# Autodesk Inventor assembly: gasienica_zlozenie
(part 2 of 2)
- [Mate]: ramie_2_wahacza:10 ↔ tuleja_TUF106040:39
- [Angle] (0 deg): ramie_2_wahacza:10 ↔ tuleja_TUF106040:39
- [Mate]: Korpus:5 ↔ Tlok:5
- [Angle] (0 deg): Korpus:5 ↔ Tlok:5
- [Mate]: Korpus:5 ↔ Nakretka:5
- [Mate] (5 mm): Korpus:5 ↔ Nakretka:5
- Walcowe:5 [CylindricalJoint]: Korpus:5 ↔ Tlok:5
- [Mate]: Korpus:5 ↔ M5_70_shaft:5
- [Flush] (-30 mm): Korpus:5 ↔ M5_70_shaft:5
- [Mate]: M5_nut_5mm:28 ↔ M5_70_shaft:5
- [Mate]: M5_70_shaft:5 ↔ M5_nut_5mm:29
- [Mate] (60 mm): M5_nut_5mm:28 ↔ M5_nut_5mm:29
- [Mate] (30 mm): Korpus:5 ↔ M5_nut_5mm:28
- [Mate]: tuleja_TUF106040:38 ↔ ramie_1_wahacza:10
- [Mate]: tuleja_TUF106040:37 ↔ ramie_1_wahacza:10
- [Mate]: tuleja_TUF106040:38 ↔ ramie_1_wahacza:10
- [Mate]: tuleja_TUF106040:33 ↔ tuleja_TUF106040:39
- [Mate]: wspornik_amortyzatora:9 ↔ wspornik_amortyzatora:10
- [Mate]: wspornik_amortyzatora:9 ↔ wspornik_amortyzatora:10
- [Mate] (5 mm): wspornik_amortyzatora:9 ↔ wspornik_amortyzatora:10
- [Mate]: M3_16_shaft:5 ↔ wspornik_amortyzatora:10
- [Flush] (-2.5 mm): M3_16_shaft:5 ↔ wspornik_amortyzatora:9
- [Mate]: M3_16_shaft:5 ↔ M3_nut_2,5mm:9
- [Mate]: M3_nut_2,5mm:9 ↔ wspornik_amortyzatora:9
- [Mate]: M3_16_shaft:5 ↔ M3_nut_2,5mm:10
- [Mate]: M3_nut_2,5mm:10 ↔ wspornik_amortyzatora:10
- [Mate]: Tlok:5 ↔ M3_16_shaft:5
- [Mate]: Tlok:5 ↔ wspornik_amortyzatora:10
- [Mate]: ramie_1_wahacza:9 ↔ wspornik_amortyzatora:9
- [Mate]: ramie_1_wahacza:9 ↔ wspornik_amortyzatora:9
- [Mate] (4.5 mm): ramie_1_wahacza:9 ↔ wspornik_amortyzatora:9
- [Mate]: tuleja_TUF106040:36 ↔ M6_40_shaft:9
- [Flush] (7 mm): ramie_1_wahacza:9 ↔ M6_40_shaft:9
- [Mate]: tuleja_TUF106040:39 ↔ M6_40_shaft:10
- [Flush] (7 mm): ramie_2_wahacza:10 ↔ M6_40_shaft:10
- [Mate]: M6_nut_5mm:41 ↔ M6_40_shaft:9
- [Mate]: ramie_1_wahacza:9 ↔ M6_nut_5mm:41
- [Mate]: M6_40_shaft:9 ↔ M6_nut_5mm:42
- [Mate]: ramie_1_wahacza:10 ↔ M6_nut_5mm:42
- [Mate]: M6_40_shaft:10 ↔ M6_nut_5mm:43
- [Mate]: ramie_2_wahacza:9 ↔ M6_nut_5mm:43
- [Mate]: M6_40_shaft:10 ↔ M6_nut_5mm:44
- [Mate]: ramie_2_wahacza:10 ↔ M6_nut_5mm:44
- [Mate]: M6_40_shaft:9 ↔ tuleja_M6_M10_7:10
- [Mate]: M6_40_shaft:10 ↔ tuleja_M6_M10_7:11
- [Mate]: M6_1,25_pad:33 ↔ M6_1,25_pad:34
- [Mate]: M6_1,25_pad:33 ↔ M6_1,25_pad:34
- [Mate]: M6_40_shaft:9 ↔ M6_1,25_pad:33
- [Mate]: M6_1,25_pad:35 ↔ M6_1,25_pad:36
- [Mate]: M6_1,25_pad:35 ↔ M6_1,25_pad:36
- [Mate]: M6_40_shaft:9 ↔ M6_1,25_pad:35
- [Mate]: tuleja_TUF106040:36 ↔ M6_1,25_pad:35
- [Mate]: M6_1,25_pad:37 ↔ M6_1,25_pad:38
- [Mate]: M6_1,25_pad:37 ↔ M6_1,25_pad:38
- [Mate]: M6_40_shaft:10 ↔ M6_1,25_pad:37
- [Mate]: M6_1,25_pad:39 ↔ M6_1,25_pad:40
- [Mate]: M6_1,25_pad:39 ↔ M6_1,25_pad:40
- [Mate]: M6_40_shaft:10 ↔ M6_1,25_pad:39
- [Mate]: tuleja_TUF106040:39 ↔ M6_1,25_pad:39
- [Mate]: M5_70_shaft:5 ↔ M6_70_shaft:9
- [Flush]: M5_70_shaft:5 ↔ M6_70_shaft:10
- [Mate]: M6_70_shaft:10 ↔ M6_nut_5mm:45
- [Mate]: M6_70_shaft:10 ↔ M6_nut_5mm:46
- [Mate] (60 mm): M6_nut_5mm:45 ↔ M6_nut_5mm:46
- [Flush]: M5_nut_5mm:28 ↔ M6_nut_5mm:46
- [Mate] (60 mm): M6_nut_5mm:47 ↔ M6_nut_5mm:48
- [Mate]: M6_nut_5mm:47 ↔ M6_nut_5mm:48
- [Mate]: M6_70_shaft:9 ↔ M6_nut_5mm:47
- [Flush]: M5_nut_5mm:28 ↔ M6_nut_5mm:48
- [Mate]: ramie_1_wahacza:9 ↔ M5_shaft:9
- [Flush] (7 mm): ramie_1_wahacza:9 ↔ M5_shaft:9
- [Mate]: ramie_1_wahacza:9 ↔ M5_shaft:10
- [Flush] (7 mm): ramie_1_wahacza:9 ↔ M5_shaft:10
- [Mate]: M5_shaft:10 ↔ M5_nut_5mm:30
- [Mate]: ramie_1_wahacza:9 ↔ M5_nut_5mm:30
- [Mate]: M5_shaft:9 ↔ M5_nut_5mm:31
- [Mate]: ramie_1_wahacza:9 ↔ M5_nut_5mm:31
- [Mate]: M5_shaft:9 ↔ M5_nut_5mm:32
- [Mate]: ramie_1_wahacza:10 ↔ M5_nut_5mm:32
- [Mate]: M5_shaft:10 ↔ M5_nut_5mm:33
- [Mate]: ramie_1_wahacza:10 ↔ M5_nut_5mm:33
- [Mate]: M5_70_shaft:5 ↔ tuleja_M5_M9_20:5
- [Mate]: Korpus:5 ↔ tuleja_M5_M9_20:5
- [Mate]: M5_70_shaft:5 ↔ tuleja_M5_M9_25:5
- [Mate]: Korpus:5 ↔ tuleja_M5_M9_25:5
- [Mate]: M5_shaft:9 ↔ tuleja_M5_M9_4,5:17
- [Mate]: ramie_1_wahacza:10 ↔ tuleja_M5_M9_4,5:17
- [Mate]: M5_shaft:9 ↔ tuleja_M5_M9_4,5:18
- [Mate]: ramie_1_wahacza:9 ↔ tuleja_M5_M9_4,5:18
- [Mate]: M5_shaft:10 ↔ tuleja_M5_M9_4,5:19
- [Mate]: ramie_1_wahacza:10 ↔ tuleja_M5_M9_4,5:19
- [Mate]: M5_shaft:10 ↔ tuleja_M5_M9_4,5:20
- [Mate]: ramie_1_wahacza:9 ↔ tuleja_M5_M9_4,5:20
- [Mate]: M6_40_shaft:10 ↔ glowny_wahacz_zewn:3
- [Mate]: tuleja_M6_M10_7:11 ↔ glowny_wahacz_zewn:3
- [Mate]: M6_40_shaft:9 ↔ glowny_wahacz_zewn:3
- [Mate]: M6_40_shaft:10 ↔ glowny_wahacz_zewn:4
- [Mate]: M6_40_shaft:9 ↔ glowny_wahacz_zewn:4
- [Mate]: tuleja_TUF106040:38 ↔ M6_40_shaft:9
- [Mate]: M6_1,25_pad:36 ↔ glowny_wahacz_zewn:4
- [Mate]: M6_1,25_pad:40 ↔ glowny_wahacz_zewn:4
- [Mate]: tuleja_M6_M10_7:10 ↔ glowny_wahacz_zewn:3
- [Mate]: M6_1,25_pad:33 ↔ glowny_wahacz_zewn:3
- [Mate]: tuleja_TUF106040:38 ↔ M6_1,25_pad:34
- [Mate]: M6_1,25_pad:37 ↔ glowny_wahacz_zewn:3
- [Mate]: tuleja_TUF106040:33 ↔ M6_1,25_pad:38
- [Mate]: tuleja_TUF106040:37 ↔ ramie_1_wahacza:10
- [Mate]: tuleja_TUF106040:35 ↔ M6_70_shaft:10
- [Mate]: ramie_1_wahacza:9 ↔ tuleja_TUF106040:35
- [Mate]: ramie_1_wahacza:9 ↔ tuleja_TUF106040:35
- [Mate]: tuleja_TUF106040:34 ↔ M6_70_shaft:9
- [Mate]: ramie_2_wahacza:9 ↔ tuleja_TUF106040:34
- [Mate]: ramie_2_wahacza:9 ↔ tuleja_TUF106040:34
- [Mate]: tuleja_TUF106040:40 ↔ M6_70_shaft:9
- [Mate]: ramie_2_wahacza:10 ↔ tuleja_TUF106040:40
- [Mate]: ramie_2_wahacza:10 ↔ tuleja_TUF106040:40
- [Mate]: M6_70_shaft:9 ↔ tuleja_M6_M10_8,5:9
- [Mate]: tuleja_TUF106040:40 ↔ tuleja_M6_M10_8,5:9
- [Mate]: M6_70_shaft:9 ↔ tuleja_M6_M10_13,5:9
- [Mate]: M6_70_shaft:10 ↔ tuleja_M6_M10_13,5:10
- [Mate]: tuleja_TUF106040:37 ↔ tuleja_M6_M10_13,5:10
- [Mate]: tuleja_TUF106040:34 ↔ tuleja_M6_M10_13,5:9
- [Mate]: M6_70_shaft:10 ↔ tuleja_M6_M10_8,5:10
- [Mate]: tuleja_TUF106040:35 ↔ tuleja_M6_M10_8,5:10
- [Mate]: independent_wheel_pair:2 ↔ tuleja_M6_M10_7:12
- [Mate]: glowny_wahacz_zewn:4 ↔ independent_wheel_pair:2
- [Mate]: glowny_wahacz_zewn:4 ↔ independent_wheel_pair:2
- [Mate]: glowny_wahacz_zewn:4 ↔ tuleja_M6_M10_7:12
- Zestawiające:1006 [Mate]: plyta_glowna_V3:2 ↔ M5_nut_5mm:28
- Zestawiające:1007 [Mate]: glowny_wahacz_zewn:3 ↔ independent_wheel_pair:2
- Zestawiające:1008 [Mate]: glowny_wahacz_zewn:3 ↔ tuleja_M6_M10_7:12
- Zestawiające:1009 [Mate]: plyta_glowna_V3:2 ↔ M6_70_shaft:10
- Zestawiające:1010 [Mate]: tuleja_TUF106040:37 ↔ M6_70_shaft:10
- Zestawiające:1011 [Mate]: plyta_glowna_V3:2 ↔ tuleja_M6_M10_13,5:9
- Zestawiające:1012 [Mate]: plyta_glowna_V3:2 ↔ tuleja_M5_M9_25:5
## Named parameters: d47_d24 = 0 mm, d48_d25 = 0 mm, d17_d47_d24 = 0 mm, d18_d48_d25 = 0 mm, d19_d15 = 0 mm, d20_d16 = 5 mm, d25_d17_d47_d24 = 0 mm, d26_d18_d48_d25 = 0 mm, d27_d19_d15 = 0 mm, d28_d20_d16 = 5 mm, d102_d31 = 0 mm, d103_d32 = 7 mm, d104_d33 = 0 mm, d105_d34 = 0 mm, d705_d35 = 0 mm, d706_d36 = 31 mm, d707_d37 = 0 mm, d109_d23 = 0 mm, d110_d24 = 0 mm, d111_d25 = 0 mm, d112_d26 = 0 mm, d113_d27 = 7 mm, d114_d28 = 0 mm, d115_d30 = 0 mm, d715_d116 = 0 mm, d716_d117 = 0 mm, d717_d118 = 0 mm, d718_d119 = 0 mm, susp_angle = 108 deg, d917_d233 = 0 mm, d918_d234 = 0 mm, d919_d235 = 0 mm, d920_d236 = 0 mm, d921_d237 = 0 mm, d922_d205 = 0 mm, d923_d206 = 0 mm, d924_d207 = 0 mm, d925_d208 = 0 mm, d926_d209 = 0 mm, d927_d210 = 0 mm, d928_d211 = 0 mm, d929_d212 = 0 mm, d930_d213 = 0 mm, d931_d214 = 0 mm, d932_d215 = 0 mm, d933_d216 = 0 mm, d934_d217 = 0 mm, d935_d218 = 0 mm, d936_d219 = 0 mm, d937_d220 = 0 mm, d938_d221 = 0 mm, d939_d222 = 0 mm, d940_d223 = 0 mm, d941_d224 = 0 mm, d942_d225 = 0 mm, d943_d226 = 0 mm, d944_d227 = 0 mm, d945_d228 = 0 mm, d946_d229 = 0 mm, d947_d230 = 0 mm, d948_d231 = 0 mm, d949_d232 = 0 mm, d950_d168 = 0 mm, d951_d169 = 0 mm, d952_d172 = 0 mm, d953_d173 = 0 mm, d954_d174 = 0 mm, d955_d175 = 0 mm, d956_d176 = 60 mm, d957_d177 = 0 mm, d958_d178_d176 = 60 mm, d959_d179 = 0 mm, d960_d180 = 0 mm, d961_d181 = 0 mm, d962_d190 = 0 mm, d963_d191 = 7 mm, d964_d192 = 0 mm, d965_d193 = 7 mm, d966_d194 = 0 mm, d967_d195 = 0 mm, d968_d196 = 0 mm, d969_d197 = 0 mm, d970_d198 = 0 mm, d971_d199 = 0 mm, d972_d200 = 0 mm, d973_d201 = 0 mm, d974_d202 = 0 mm, d975_d203 = 0 mm, d976_d204 = 0 mm, d977_d136 = 0 mm, d978_d137 = 4.5 mm, d979_d138 = 0 mm, d980_d139 = 7 mm, d981_d140 = 0 mm, d982_d141 = 7 mm, d983_d142 = 0 mm, d984_d143 = 0 mm, d985_d144 = 0 mm, d986_d145 = 0 mm, d987_d146 = 0 mm, d988_d147 = 0 mm, d989_d148 = 0 mm, d990_d149 = 0 mm, d991_d150 = 0 mm, d992_d151 = 0 mm, d993_d152 = 0 mm, d994_d153 = 0 mm, d995_d154 = 0 mm, d996_d155 = 0 mm, d997_d156 = 0 mm, d998_d157 = 0 mm, d999_d158_d154 = 0 mm, d1000_d159_d155 = 0 mm, d1001_d160 = 0 mm, d1002_d161 = 0 mm, d1003_d162_d154 = 0 mm, d1004_d163_d155 = 0 mm, d1005_d164 = 0 mm, d1006_d165 = 0 mm, d1007_d166_d154 = 0 mm, d1008_d167_d155 = 0 mm, d1009_d106 = 0 mm, d1010_d107 = 0 mm, d1011_d108 = 0 mm, d1012_d109 = -30 mm, d1013_d110 = 0 mm, d1014_d111 = 0 mm, d1015_d112 = 60 mm, d1016_d113 = 30 mm, d1017_d114 = 0 mm, d1018_d116 = 0 mm, d1019_d118 = 0 mm, d1020_d119 = 0 mm, d1021_d120 = 0 mm, d1022_d121 = 0 mm, d1023_d122 = 5 mm, d1024_d123 = 0 mm, d1025_d124 = -2.5 mm, d1026_d125 = 0 mm, d1027_d126 = 0 mm, d1028_d127 = 0 mm, d1029_d128 = 0 mm, d1030_d129 = 0 mm, d1031_d130 = 0 mm, d1032_d131 = 0 mm, d1033_d132 = 2.5 mm, d1034_d133 = 2.5 mm, d1035_d134 = 0 mm, d1036_d135 = 0 mm, d1037_d10 = 0 mm, d1038_d11 = 0 deg, d1039_d22 = 0 mm, d1040_d23 = 0 mm, d1041_d24 = 0 mm, d1042_d25 = 0 mm, d1043_d38 = 2.5 mm, d1044_d41_d4 = 0 deg, d1045_d43_d0 = 0 mm, d1046_d44_d1 = 0 mm, d1047_d46 = 2.5 mm, d1048_d52 = 0 mm, d1049_d83_d6 = 1 mm, d1050_d84_d7 = -2 mm, d1051_d85_d8 = -13 mm, d1052_d86_d0 = 0 mm, d1053_d87_d1 = 0 deg, d1054_d88_d3 = 0 mm, d1055_d89_d4 = 5 mm, d1056_d90_d5 = 0 deg, d1057_d103 = 0 mm, d1058_d104 = 0 mm, d1059_d105 = 6 mm, d1060_d0 = 0 mm, d1061_d1 = 0 mm, d1062_d4 = 0 deg, d1063_d9 = 0 mm, d1076_d208 = 0 mm, d1077_d209 = 0 mm, d1078_d210 = 0 mm, d1080_d212 = 0 mm, d178_d176 = 60 mm, d158_d154 = 0 mm, d159_d155 = 0 mm, d162_d154 = 0 mm, d163_d155 = 0 mm, d166_d154 = 0 mm, d167_d155 = 0 mm, d1189_d11 = 0 deg, d1190_d22 = 0 mm, d1191_d23 = 0 mm, d1192_d24 = 0 mm, d41_d4 = 0 deg, d43_d0 = 0 mm, d44_d1 = 0 mm, d83_d6 = 1 mm, d84_d7 = -6.4534 mm, d85_d8 = -13 mm, d86_d0 = 0 mm, d87_d1 = 0 deg, d88_d3 = 0 mm, d89_d4 = 5 mm, d90_d5 = 0 deg, d1211_d0 = 0 mm, d1212_d1 = 0 mm, d1219_d0 = 0 mm, d1220_d1 = 0 mm, d1221_d4 = 0 deg, d1222_d9 = 0 mm, d1228_d221 = 0 mm, d1229_d222 = 0 mm, d1232_d225 = 0 mm, d1238_d231 = 0 mm, d1239_d232 = 0 mm, d1240_d233 = 0 mm, d1241_d234 = 0 mm, d1242_d235 = 0 mm, d1243_d236 = 0 mm, d1244_d237 = 0 mm, d1258_d191 = 7 mm, d1259_d192 = 0 mm, d1260_d193 = 7 mm, d1261_d194 = 0 mm, d1262_d195 = 0 mm, d1263_d196 = 0 mm, d1264_d197 = 0 mm, d1265_d198 = 0 mm, d1266_d199 = 0 mm, d1267_d200 = 0 mm, d1268_d201 = 0 mm, d1269_d202 = 0 mm, d1270_d203 = 0 mm, d1271_d204 = 0 mm, d1272_d205 = 0 mm, d1273_d206 = 0 mm, d1274_d207 = 0 mm, d1275_d208 = 0 mm, d1276_d209 = 0 mm, d1277_d210 = 0 mm, d1278_d211 = 0 mm, d1279_d212 = 0 mm, d1280_d213 = 0 mm, d1281_d216 = 0 mm, d1282_d217 = 0 mm, d1283_d218 = 0 mm, d1286_d149 = 0 mm, d1287_d150 = 0 mm, d1288_d152 = 0 mm, d1289_d154 = 0 mm, d1290_d155 = 0 mm, d1291_d156 = 0 mm, d1292_d158_d154 = 0 mm, d1293_d159_d155 = 0 mm, d1294_d160 = 0 mm, d1295_d161 = 0 mm, d1296_d162_d154 = 0 mm, d1297_d163_d155 = 0 mm, d1298_d164 = 0 mm, d1299_d166_d154 = 0 mm, d1300_d167_d155 = 0 mm, d1301_d168 = 0 mm, d1302_d169 = 0 mm, d1303_d172 = 0 mm, d1304_d173 = 0 mm, d1305_d174 = 0 mm, d1306_d175 = 0 mm, d1307_d176 = 60 mm, d1308_d177 = 0 mm, d1309_d178_d176 = 60 mm, d1310_d179 = 0 mm, d1311_d180 = 0 mm, d1312_d181 = 0 mm, d1313_d190 = 0 mm, d1314_d113 = 30 mm, d1315_d114 = 0 mm, d1317_d116 = 0 mm, d1318_d119 = 0 mm, d1319_d120 = 0 mm, d1320_d121 = 0 mm, d1321_d122 = 5 mm, d1322_d123 = 0 mm, d1323_d124 = -2.5 mm, d1324_d125 = 0 mm, d1325_d126 = 0 mm, d1326_d127 = 0 mm, d1327_d128 = 0 mm, d1328_d129 = 0 mm, d1329_d130 = 0 mm, d1330_d135 = 0 mm, d1331_d136 = 0 mm, d1332_d137 = 4.5 mm, d1333_d138 = 0 mm, d1334_d139 = 7 mm, d1335_d140 = 0 mm, d1336_d141 = 7 mm, d1337_d142 = 0 mm, d1338_d143 = 0 mm, d1339_d144 = 0 mm, d1340_d145 = 0 mm, d1341_d146 = 0 mm, d1342_d147 = 0 mm, d1343_d148 = 0 mm, d1344_d10 = 0 mm, d1345_d11 = 0 deg, d1346_d41_d4 = 0 deg, d1347_d43_d0 = 0 mm, d1348_d44_d1 = 0 mm, d1349_d83_d6 = 1 mm, d1350_d84_d7 = -7.2041 mm, d1351_d85_d8 = -13 mm, d1352_d86_d0 = 0 mm, d1353_d87_d1 = 0 deg, d1354_d88_d3 = 0 mm, d1355_d89_d4 = 5 mm, d1356_d90_d5 = 0 deg, d1358_d108 = 0 mm, d1359_d109 = -30 mm, d1360_d110 = 0 mm, d1361_d111 = 0 mm, d1362_d112 = 60 mm, d1371_d233 = 0 mm, d1372_d234 = 0 mm, d1373_d235 = 0 mm, d1374_d236 = 0 mm, d1375_d237 = 0 mm, d1376_d238 = 0 mm, d1377_d239 = 0 mm, d1378_d240 = 0 mm, d1379_d241 = 0 mm, d1380_d242 = 0 mm, d1381_d243 = 0 mm, d1382_d244 = 0 mm, d1383_d245 = 0 mm, d1384_d246 = 0 mm, d1385_d247 = 0 mm, d1386_d250 = 0 mm, d1387_d251 = 0 mm, d1388_d252 = 0 mm, d1389_d254 = 0 mm, d1390_d255 = 0 mm, d1391_d256 = 0 mm, d1392_d257 = 0 mm, d1393_d258 = 0 mm, d1394_d1369 = 0 mm, d1398_d195 = 0 mm, d1399_d196 = 0 mm, d1400_d197 = 0 mm, d1401_d198 = 0 mm, d1402_d199 = 0 mm, d1403_d200 = 0 mm, d1404_d201 = 0 mm, d1405_d202 = 0 mm, d1406_d203 = 0 mm, d1407_d204 = 0 mm, d1408_d205 = 0 mm, d1409_d206 = 0 mm, d1410_d207 = 0 mm, d1411_d208 = 0 mm, d1412_d209 = 0 mm, d1413_d210 = 0 mm, d1414_d211 = 0 mm, d1415_d212 = 0 mm, d1416_d213 = 0 mm, d1417_d216 = 0 mm, d1418_d217 = 0 mm, d1419_d218 = 0 mm, d1420_d221 = 0 mm, d1421_d222 = 0 mm, d1422_d225 = 0 mm, d1423_d231 = 0 mm, d1424_d232 = 0 mm, d1425_d154 = 0 mm, d1426_d155 = 0 mm, d1427_d156 = 0 mm, d1428_d158_d154 = 0 mm, d1429_d159_d155 = 0 mm, d1430_d160 = 0 mm, d1431_d161 = 0 mm, d1432_d162_d154 = 0 mm, d1433_d163_d155 = 0 mm, d1434_d164 = 0 mm, d1435_d166_d154 = 0 mm, d1436_d167_d155 = 0 mm, d1437_d168 = 0 mm, d1438_d169 = 0 mm, d1439_d172 = 0 mm, d1440_d173 = 0 mm, d1441_d174 = 0 mm, d1442_d175 = 0 mm, d1443_d176 = 60 mm, d1444_d177 = 0 mm, d1445_d178_d176 = 60 mm, d1446_d179 = 0 mm, d1447_d180 = 0 mm, d1448_d181 = 0 mm, d1449_d190 = 0 mm, d1450_d191 = 7 mm, d1451_d192 = 0 mm, d1452_d193 = 7 mm, d1453_d194 = 0 mm, d1454_d119 = 0 mm, d1455_d120 = 0 mm, d1456_d121 = 0 mm, d1457_d122 = 5 mm, d1458_d123 = 0 mm, d1459_d124 = -2.5 mm, d1460_d125 = 0 mm, d1461_d126 = 0 mm, d1462_d127 = 0 mm, d1463_d128 = 0 mm, d1464_d129 = 0 mm, d1465_d130 = 0 mm, d1466_d135 = 0 mm, d1467_d136 = 0 mm, d1468_d137 = 4.5 mm, d1469_d138 = 0 mm, d1470_d139 = 7 mm, d1471_d140 = 0 mm, d1472_d141 = 7 mm, d1473_d142 = 0 mm, d1474_d143 = 0 mm, d1475_d144 = 0 mm, d1476_d145 = 0 mm, d1477_d146 = 0 mm, d1478_d147 = 0 mm, d1479_d148 = 0 mm, d1480_d149 = 0 mm, d1481_d150 = 0 mm, d1482_d152 = 0 mm, d1483_d10 = 0 mm, d1484_d11 = 0 deg, d1485_d41_d4 = 0 deg, d1486_d43_d0 = 0 mm, d1487_d44_d1 = 0 mm, d1488_d83_d6 = 1 mm, d1489_d84_d7 = -4.5901 mm, d1490_d85_d8 = -13 mm, d1491_d86_d0 = 0 mm, d1492_d87_d1 = 0 deg, d1493_d88_d3 = 0 mm, d1494_d89_d4 = 5 mm, d1495_d90_d5 = 0 deg, d1496_d108 = 0 mm, d1497_d109 = -30 mm, d1498_d110 = 0 mm, d1499_d111 = 0 mm, d1500_d112 = 60 mm, d1501_d113 = 30 mm, d1502_d114 = 0 mm, d1503_d115 = 0 mm, d1504_d116 = 0 mm, d1505_d0 = 0 mm, d1506_d1 = 0 mm, d1507_d4 = 0 deg, d1508_d9 = 0 mm, tlok_scisniety = -13 mm, tlok_wyprostowany = 1 mm
